# Autodesk Inventor assembly: Mecanismo Modelado
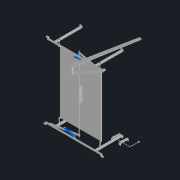
[picture p0: Inventor's stored thumbnail of the model, 180x180]
Saved by Autodesk Inventor 2021 (Build 250183000, 183)
## iProperties
Created: 2021-04-19
Part Number: Mecanismo Modelado
Document SubType Name: Assembly
Designer: carlo
Author: carlo
## Documents named in this file (18)
- J:\PAI\Proyecto_PAI_2021\01 CAD\Mecanismo Modelado.iam
- J:\PAI\Proyecto_PAI_2021\01 CAD\Bancada.ipt
- J:\PAI\Proyecto_PAI_2021\01 CAD\Eslabon1.ipt
- J:\PAI\Proyecto_PAI_2021\01 CAD\Eslabon2.ipt
- J:\PAI\Proyecto_PAI_2021\01 CAD\Palanca.ipt
- J:\PAI\Proyecto_PAI_2021\01 CAD\pin10.ipt
- J:\PAI\Proyecto_PAI_2021\01 CAD\union.ipt
- J:\PAI\Proyecto_PAI_2021\01 CAD\Bandeja.ipt
- J:\PAI\Proyecto_PAI_2021\01 CAD\Pincerrado.ipt
- J:\PAI\Proyecto_PAI_2021\01 CAD\PinCorto.ipt
- J:\PAI\Proyecto_PAI_2021\01 CAD\PinLargo.ipt
- J:\PAI\Proyecto_PAI_2021\01 CAD\arandela.ipt
- J:\PAI\Proyecto_PAI_2021\01 CAD\MecanismoBoqueoCarro\CilindroAjuste.ipt
- J:\PAI\Proyecto_PAI_2021\01 CAD\MecanismoBoqueoCarro\Fijador.ipt
- J:\PAI\Proyecto_PAI_2021\01 CAD\MecanismoBoqueoCarro\UnionOrtogonal.ipt
- J:\PAI\Proyecto_PAI_2021\01 CAD\MecanismoBoqueoCarro\PistaSistBloq.ipt
- J:\PAI\Proyecto_PAI_2021\01 CAD\MecanismoBoqueoCarro\Barra en L.ipt
- J:\PAI\Proyecto_PAI_2021\01 CAD\MecanismoBoqueoCarro\FijadorParaBloqueo.ipt
## Components (35 placed, 17 different names)
1. Bancada:1 — Coincidencia:1, Nivelación:15, Coincidencia:7, Nivelación:16, Tangente:14, Cilíndrica:26, Coincidencia:60, Tangente:15, Tangente:16, Nivelación:30, Coincidencia:66
2. Eslabon1:1 — Coincidencia:1, Coincidencia:2, Cilíndrica:19, Coincidencia:9, Cilíndrica:27
3. Eslabon2:1 — Coincidencia:2, Coincidencia:3, Cilíndrica:18, Coincidencia:8, Cilíndrica:25, Cilíndrica:29, Nivelación:29, Coincidencia:64
4. Palanca:1 — Coincidencia:3, Coincidencia:4, Nivelación:5, Coincidencia:13
5. pin10:1 — Coincidencia:4, Nivelación:5
6. Bancada:2 — Nivelación:15, Coincidencia:7, Nivelación:16, Coincidencia:11, Flush:21, Mate:31, Mate:32, Mate:40, Tangent:13, Cilíndrica:28
7. Eslabon1:2 — Coincidencia:6, Cilíndrica:20, Coincidencia:11, Coincidencia:14, Mate:57
8. Eslabon2:2 — Coincidencia:6, Cilíndrica:21, Coincidencia:10, Coincidencia:15, Mate:59, Cilíndrica:30, Coincidencia:62
9. union:1 — Cilíndrica:29, Cilíndrica:30, Nivelación:29, Coincidencia:61, Coincidencia:63, Cilíndrica:31
10. Bandeja:1 — Cilíndrica:31, Tangente:15, Tangente:16, Nivelación:30, Coincidencia:65, Coincidencia:67, Coincidencia:68, Coincidencia:69, Coincidencia:70, Coincidencia:71, Coincidencia:72
11. Pincerrado:1 — Cilíndrica:18, Coincidencia:8, Cilíndrica:19, Coincidencia:9
12. Pincerrado:2 — Cilíndrica:20, Cilíndrica:21, Coincidencia:10
13. PinCorto:1 — Cilíndrica:26, Cilíndrica:27, Coincidencia:60
14. PinLargo:1 — Cilíndrica:25, Coincidencia:13, Tangente:14
15. PinCorto:2 — Coincidencia:14, Mate:57, Cilíndrica:28
16. Pincerrado:3 — Coincidencia:15, Tangent:13, Mate:59
17. arandela:1 — Coincidencia:65, Coincidencia:66
18. arandela:2 — Coincidencia:63, Coincidencia:64
19. arandela:3 — Coincidencia:67, Coincidencia:68
20. arandela:4 — Coincidencia:69, Coincidencia:70
21. arandela:5 — Coincidencia:61, Coincidencia:62
22. arandela:6 — Coincidencia:71, Coincidencia:72
23. CilindroAjuste:1 — Mate:28, Mate:29, Mate:30, Tangent:9
24. Fijador:1 — Mate:29
25. UnionOrtogonal:1 — Mate:28, Mate:34, Flush:26, Mate:51, Mate:53
26. Fijador:2 — Mate:30, Mate:33
27. PistaSistBloq:1 — Flush:21, Mate:31, Tangent:9, Mate:32, Mate:33, Mate:34, Flush:23, Flush:24, Flush:25, Flush:26
28. Fijador:3 — Mate:48, Flush:28, Mate:51
29. FijadorParaBloqueo:1 — Mate:50, Mate:52
30. PistaSistBloq:2 — Flush:23, Flush:24, Flush:25, Mate:40, Tangent:10, Mate:45, Flush:27, Angle:1
31. Fijador:4 — Mate:41, Mate:45
32. CilindroAjuste:2 — Mate:41, Mate:42, Mate:43, Tangent:10
33. UnionOrtogonal:2 — Mate:43, Mate:44, Flush:27, Mate:54
34. Fijador:5 — Mate:42, Mate:44
35. Barra en L:1 — Mate:48, Mate:50, Flush:28, Mate:52, Angle:1, Mate:53, Mate:54
## Relationships (77: Mate 47, Flush 12, CylindricalJoint 11, Tangent 6, Angle 1)
- Coincidencia:1 [Mate] (10 mm): Bancada:1 ↔ Eslabon1:1
- Coincidencia:2 [Mate] (3 mm): Eslabon1:1 ↔ Eslabon2:1
- Coincidencia:3 [Mate] (10 mm): Eslabon2:1 ↔ Palanca:1
- Coincidencia:4 [Mate]: Palanca:1 ↔ pin10:1
- Nivelación:5 [Flush]: Palanca:1 ↔ pin10:1
- Coincidencia:6 [Mate] (3 mm): Eslabon1:2 ↔ Eslabon2:2
- Nivelación:15 [Flush]: Bancada:1 ↔ Bancada:2
- Coincidencia:7 [Mate] (-507.58 mm): Bancada:1 ↔ Bancada:2
- Nivelación:16 [Flush]: Bancada:1 ↔ Bancada:2
- Cilíndrica:18 [CylindricalJoint]: Eslabon2:1 ↔ Pincerrado:1
- Coincidencia:8 [Mate]: Eslabon2:1 ↔ Pincerrado:1
- Cilíndrica:19 [CylindricalJoint]: Eslabon1:1 ↔ Pincerrado:1
- Coincidencia:9 [Mate]: Eslabon1:1 ↔ Pincerrado:1
- Cilíndrica:20 [CylindricalJoint]: Eslabon1:2 ↔ Pincerrado:2
- Cilíndrica:21 [CylindricalJoint]: Eslabon2:2 ↔ Pincerrado:2
- Coincidencia:10 [Mate]: Eslabon2:2 ↔ Pincerrado:2
- Coincidencia:11 [Mate] (-20 mm): Bancada:2 ↔ Eslabon1:2
- Cilíndrica:25 [CylindricalJoint]: Eslabon2:1 ↔ PinLargo:1
- Coincidencia:13 [Mate]: Palanca:1 ↔ PinLargo:1
- Coincidencia:14 [Mate]: Eslabon1:2 ↔ PinCorto:2
- Coincidencia:15 [Mate]: Eslabon2:2 ↔ Pincerrado:3
- Mate:28: CilindroAjuste:1 ↔ UnionOrtogonal:1
- Mate:29: CilindroAjuste:1 ↔ Fijador:1
- Mate:30: CilindroAjuste:1 ↔ Fijador:2
- Flush:21: Bancada:2 ↔ PistaSistBloq:1
- Mate:31: Bancada:2 ↔ PistaSistBloq:1
- Tangent:9: CilindroAjuste:1 ↔ PistaSistBloq:1
- Mate:32: Bancada:2 ↔ PistaSistBloq:1
- Mate:33: Fijador:2 ↔ PistaSistBloq:1
- Mate:34: UnionOrtogonal:1 ↔ PistaSistBloq:1
- Flush:23: PistaSistBloq:1 ↔ PistaSistBloq:2
- Flush:24: PistaSistBloq:1 ↔ PistaSistBloq:2
- Flush:25: PistaSistBloq:1 ↔ PistaSistBloq:2
- Mate:40 (25 mm): Bancada:2 ↔ PistaSistBloq:2
- Mate:41: Fijador:4 ↔ CilindroAjuste:2
- Mate:42: CilindroAjuste:2 ↔ Fijador:5
- Mate:43: CilindroAjuste:2 ↔ UnionOrtogonal:2
- Mate:44: UnionOrtogonal:2 ↔ Fijador:5
- Tangent:10: PistaSistBloq:2 ↔ CilindroAjuste:2
- Mate:45: PistaSistBloq:2 ↔ Fijador:4
- Flush:26 (3.75 mm): UnionOrtogonal:1 ↔ PistaSistBloq:1
- Flush:27 (3.75 mm): PistaSistBloq:2 ↔ UnionOrtogonal:2
- Mate:48: Fijador:3 ↔ Barra en L:1
- Mate:50: FijadorParaBloqueo:1 ↔ Barra en L:1
- Flush:28: Fijador:3 ↔ Barra en L:1
- Mate:51: UnionOrtogonal:1 ↔ Fijador:3
- Mate:52: FijadorParaBloqueo:1 ↔ Barra en L:1
- Angle:1 (0 deg): PistaSistBloq:2 ↔ Barra en L:1
- Mate:53: UnionOrtogonal:1 ↔ Barra en L:1
- Mate:54: UnionOrtogonal:2 ↔ Barra en L:1
- Tangent:13: Bancada:2 ↔ Pincerrado:3
- Mate:57: Eslabon1:2 ↔ PinCorto:2
- Mate:59: Eslabon2:2 ↔ Pincerrado:3
- Tangente:14: Bancada:1 ↔ PinLargo:1
- Cilíndrica:26 [CylindricalJoint]: Bancada:1 ↔ PinCorto:1
- Cilíndrica:27 [CylindricalJoint]: Eslabon1:1 ↔ PinCorto:1
- Coincidencia:60 [Mate]: Bancada:1 ↔ PinCorto:1
- Cilíndrica:28 [CylindricalJoint]: Bancada:2 ↔ PinCorto:2
- Cilíndrica:29 [CylindricalJoint]: Eslabon2:1 ↔ union:1
- Cilíndrica:30 [CylindricalJoint]: Eslabon2:2 ↔ union:1
- Nivelación:29 [Flush]: Eslabon2:1 ↔ union:1
- Coincidencia:61 [Mate]: union:1 ↔ arandela:5
- Coincidencia:62 [Mate]: Eslabon2:2 ↔ arandela:5
- Coincidencia:63 [Mate]: union:1 ↔ arandela:2
- Coincidencia:64 [Mate]: Eslabon2:1 ↔ arandela:2
- Cilíndrica:31 [CylindricalJoint]: union:1 ↔ Bandeja:1
- Tangente:15: Bancada:1 ↔ Bandeja:1
- Tangente:16: Bancada:1 ↔ Bandeja:1
- Nivelación:30 [Flush]: Bancada:1 ↔ Bandeja:1
- Coincidencia:65 [Mate]: Bandeja:1 ↔ arandela:1
- Coincidencia:66 [Mate]: Bancada:1 ↔ arandela:1
- Coincidencia:67 [Mate]: Bandeja:1 ↔ arandela:3
- Coincidencia:68 [Mate]: Bandeja:1 ↔ arandela:3
- Coincidencia:69 [Mate]: Bandeja:1 ↔ arandela:4
- Coincidencia:70 [Mate]: Bandeja:1 ↔ arandela:4
- Coincidencia:71 [Mate]: Bandeja:1 ↔ arandela:6
- Coincidencia:72 [Mate]: Bandeja:1 ↔ arandela:6
